# Autodesk Inventor assembly: DELL_PA-1131-02D2
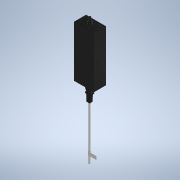
[picture p0: Inventor's stored thumbnail of the model, 180x180]
Saved by Autodesk Inventor 2021 (Build 250183000, 183)
## iProperties
Created: 2021-12-21
Part Number: DELL_PA-1131-02D2
Document SubType Name: Assembly
Designer: Jorian Brusind
Author: Jorian Brusind
## Documents named in this file (3)
- C:\Users\Jorian Brusind\Documents\GitHub\PersonalProjects\HyperRail\Inventor Files\DELL_PA-1131-02D2.iam
- C:\Users\Jorian Brusind\Documents\GitHub\PersonalProjects\HyperRail\Inventor Files\DELL_PA-1131-02D2_base.ipt
- C:\Users\Jorian Brusind\Documents\GitHub\PersonalProjects\HyperRail\Inventor Files\11-00055.iam
## Components (2 placed, 2 different names)
1. DELL_PA-1131-02D2_base:1 — Mate:1, Flush:1, Flush:2
2. 11-00055:1 [sub-assembly] — Mate:1, Flush:1, Flush:2
## Relationships (3: Flush 2, Mate 1)
- Mate:1: DELL_PA-1131-02D2_base:1 ↔ 11-00055:1
- Flush:1 (32.5 mm): DELL_PA-1131-02D2_base:1 ↔ 11-00055:1
- Flush:2 (19 mm): DELL_PA-1131-02D2_base:1 ↔ 11-00055:1
